# Autodesk Inventor assembly: Drivetrain Assembled
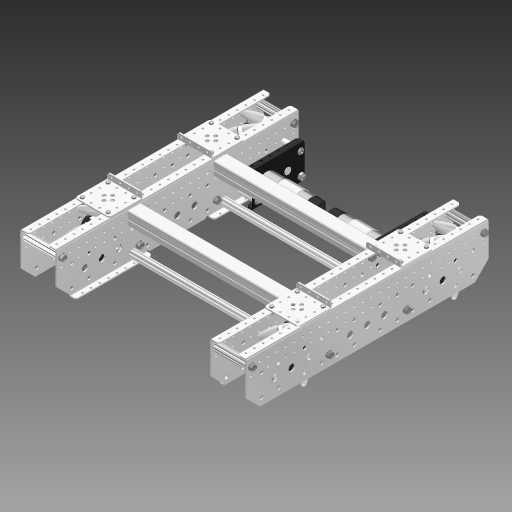
[picture p0: Inventor's stored thumbnail of the model, 512x512]
Saved by Autodesk Inventor 2024 (Build 280153000, 153)
## iProperties
Created: 2023-11-08
Part Number: Drivetrain Assembled
Document SubType Name: Assembly
Designer: Calvin
Author: Calvin
## Documents named in this file (25)
- C:\Users\Calvin\Desktop\CAD\Alt\ironChefsCAD\Drivetrain\Drivetrain Assembled.iam
- C:\Users\Calvin\Desktop\CAD\Alt\ironChefsCAD\Drivetrain\Parts\TileRunner 17 Inside Plate.ipt
- C:\Users\Calvin\Desktop\CAD\Alt\ironChefsCAD\Drivetrain\Parts\TileRunner 17 Outside Plate.ipt
- C:\Users\Calvin\Desktop\CAD\Alt\ironChefsCAD\Drivetrain\Parts\63mm Churro.ipt
- C:\Users\Calvin\Desktop\CAD\Alt\ironChefsCAD\Drivetrain\Parts\FHTS 0.25-20-0.75_FHTS 0.25-20-G-0.75-C.ipt
- C:\Users\Calvin\Desktop\CAD\Alt\ironChefsCAD\Drivetrain\Parts\TileRunner 17 4x4 Hole Bracket.ipt
- C:\Users\Calvin\Desktop\CAD\Alt\ironChefsCAD\Drivetrain\Parts\6-32 Nylock Nut_90631A007.ipt
- C:\Users\Calvin\Desktop\CAD\Alt\ironChefsCAD\Drivetrain\Parts\6-32 x 0500 HHCS_93075A148.ipt
- C:\Users\Calvin\Desktop\CAD\Alt\ironChefsCAD\Drivetrain\Parts\11.250in Peanut.ipt
- C:\Users\Calvin\Desktop\CAD\Alt\ironChefsCAD\Drivetrain\Parts\11.250in Churro.ipt
- C:\Users\Calvin\Desktop\CAD\Alt\ironChefsCAD\Drivetrain\Parts\PicoBox Uno Plate.ipt
- C:\Users\Calvin\Desktop\CAD\Alt\ironChefsCAD\Drivetrain\Parts\PicoBox Spacer.ipt
- C:\Users\Calvin\Desktop\CAD\Alt\ironChefsCAD\Drivetrain\Parts\14-20 x 1.625 BHCS_92949A837.ipt
- C:\Users\Calvin\Desktop\CAD\Alt\ironChefsCAD\Drivetrain\Parts\14-20 NyLock thin - Mcm 90566A029_90566A029.ipt
- C:\Users\Calvin\Desktop\CAD\Alt\ironChefsCAD\Drivetrain\Parts\6mm x 12mm Flanged -Mcm 7804K142_7804K142.ipt
- C:\Users\Calvin\Desktop\CAD\Alt\ironChefsCAD\Drivetrain\Parts\6mm D-Shaft 100mm.ipt
- C:\Users\Calvin\Desktop\CAD\Alt\ironChefsCAD\Drivetrain\Parts\am-2964 NeveRest.ipt
- C:\Users\Calvin\Desktop\CAD\Alt\ironChefsCAD\Drivetrain\Parts\40T 32DP 20PA With 6mm Bore Nub Gear.ipt
- C:\Users\Calvin\Desktop\CAD\Alt\ironChefsCAD\Drivetrain\Parts\am-3215 6mmD Double Boss Nub.ipt
- C:\Users\Calvin\Desktop\CAD\Alt\ironChefsCAD\Drivetrain\Parts\10-32 x 0.25 Set Screw Cup Point.ipt
- C:\Users\Calvin\Desktop\CAD\Alt\ironChefsCAD\Drivetrain\Parts\M3x0.5x6mm SHCS_91290A111.ipt
- C:\Users\Calvin\Desktop\CAD\Alt\ironChefsCAD\Drivetrain\Parts\406 right wheel.iam
- C:\Users\Calvin\Desktop\CAD\Alt\ironChefsCAD\Drivetrain\Parts\6-32 x 1250 HHCS_93075A544.ipt
- C:\Users\Calvin\Desktop\CAD\Alt\ironChefsCAD\Drivetrain\Parts\9mmt x 6.15mm ID Aluminum Spacer AluminumSpacers.com MAS13-6-9.ipt
- C:\Users\Calvin\Desktop\CAD\Alt\ironChefsCAD\Drivetrain\Parts\.594t x .257 ID Aluminum Spacer AluminumSpacers.com AS38-14-38.ipt
## Components (158 placed, 24 different names)
1. TileRunner 17 Inside Plate:1 — Insert:4, Angle:1, Flush:2, Symmetry:1, Insert:67, Angle:3, Insert:73, Insert:119, Angle:5
2. TileRunner 17 Outside Plate:1 — Insert:3, Angle:1, Insert:11, Insert:12, Insert:13, Flush:1, Insert:145, Insert:148
3. 63mm Churro:1 — Insert:1, Insert:2, Insert:3, Insert:4
4. FHTS 0.25-20-0.75_FHTS 0.25-20-G-0.75-C:1 — Insert:1
5. FHTS 0.25-20-0.75_FHTS 0.25-20-G-0.75-C:2 — Insert:2
6. 63mm Churro:2 — Insert:11
7. FHTS 0.25-20-0.75_FHTS 0.25-20-G-0.75-C:3
8. FHTS 0.25-20-0.75_FHTS 0.25-20-G-0.75-C:4
9. 63mm Churro:3 — Insert:12
10. FHTS 0.25-20-0.75_FHTS 0.25-20-G-0.75-C:5
11. FHTS 0.25-20-0.75_FHTS 0.25-20-G-0.75-C:6
12. 63mm Churro:4 — Insert:13
13. FHTS 0.25-20-0.75_FHTS 0.25-20-G-0.75-C:7
14. FHTS 0.25-20-0.75_FHTS 0.25-20-G-0.75-C:8
15. TileRunner 17 Inside Plate:2 — Flush:2, Symmetry:1, Insert:68, Angle:4, Mate:5, Insert:74, Insert:120, Angle:6
16. TileRunner 17 Outside Plate:2 — Flush:1, Flush:12, Mate:2, Mate:3, Mate:4, Insert:146, Insert:147
17. 63mm Churro:5
18. FHTS 0.25-20-0.75_FHTS 0.25-20-G-0.75-C:9
19. FHTS 0.25-20-0.75_FHTS 0.25-20-G-0.75-C:10
20. 63mm Churro:6
21. FHTS 0.25-20-0.75_FHTS 0.25-20-G-0.75-C:11
22. FHTS 0.25-20-0.75_FHTS 0.25-20-G-0.75-C:12
23. 63mm Churro:7
24. FHTS 0.25-20-0.75_FHTS 0.25-20-G-0.75-C:13
25. FHTS 0.25-20-0.75_FHTS 0.25-20-G-0.75-C:14
26. 63mm Churro:8
27. FHTS 0.25-20-0.75_FHTS 0.25-20-G-0.75-C:15
28. FHTS 0.25-20-0.75_FHTS 0.25-20-G-0.75-C:16
29. TileRunner 17 4x4 Hole Bracket:1 — Insert:31, Insert:32, Insert:33, Insert:34, Flush:3, Flush:5, Flush:9, Symmetry:3
30. 6-32 Nylock Nut_90631A007:1 — Insert:27
31. 6-32 x 0500 HHCS_93075A148:1 — Insert:27, Insert:31
32. 6-32 Nylock Nut_90631A007:2
33. 6-32 x 0500 HHCS_93075A148:2 — Insert:32
34. 6-32 Nylock Nut_90631A007:3
35. 6-32 x 0500 HHCS_93075A148:3 — Insert:33
36. 6-32 Nylock Nut_90631A007:4
37. 6-32 x 0500 HHCS_93075A148:4 — Insert:34
38. TileRunner 17 4x4 Hole Bracket:2 — Flush:3, Flush:5, Flush:7, Flush:8, Symmetry:2, Mate:3, Mate:4, Symmetry:3
39. 6-32 Nylock Nut_90631A007:5
40. 6-32 x 0500 HHCS_93075A148:5
41. 6-32 Nylock Nut_90631A007:6
42. 6-32 x 0500 HHCS_93075A148:6
43. 6-32 Nylock Nut_90631A007:7
44. 6-32 x 0500 HHCS_93075A148:7
45. 6-32 Nylock Nut_90631A007:8
46. 6-32 x 0500 HHCS_93075A148:8
47. TileRunner 17 4x4 Hole Bracket:3 — Flush:4, Flush:6, Flush:9
48. 6-32 Nylock Nut_90631A007:9
49. 6-32 x 0500 HHCS_93075A148:9
50. 6-32 Nylock Nut_90631A007:10
51. 6-32 x 0500 HHCS_93075A148:10
52. 6-32 Nylock Nut_90631A007:11
53. 6-32 x 0500 HHCS_93075A148:11
54. 6-32 Nylock Nut_90631A007:12
55. 6-32 x 0500 HHCS_93075A148:12
56. TileRunner 17 4x4 Hole Bracket:4 — Flush:4, Flush:6, Flush:7, Flush:8, Symmetry:2
57. 6-32 Nylock Nut_90631A007:13
58. 6-32 x 0500 HHCS_93075A148:13
59. 6-32 Nylock Nut_90631A007:14
60. 6-32 x 0500 HHCS_93075A148:14
61. 6-32 Nylock Nut_90631A007:15
62. 6-32 x 0500 HHCS_93075A148:15
63. 6-32 Nylock Nut_90631A007:16
64. 6-32 x 0500 HHCS_93075A148:16
65. FHTS 0.25-20-0.75_FHTS 0.25-20-G-0.75-C:17 — Insert:59
66. FHTS 0.25-20-0.75_FHTS 0.25-20-G-0.75-C:18 — Insert:60
67. 11.250in Peanut:1 — Insert:59, Insert:60, Insert:61, Insert:62, Insert:67, Angle:3, Mate:5
68. FHTS 0.25-20-0.75_FHTS 0.25-20-G-0.75-C:19 — Insert:62
69. FHTS 0.25-20-0.75_FHTS 0.25-20-G-0.75-C:20 — Insert:61
70. FHTS 0.25-20-0.75_FHTS 0.25-20-G-0.75-C:21
71. FHTS 0.25-20-0.75_FHTS 0.25-20-G-0.75-C:22
72. 11.250in Peanut:2 — Insert:68, Angle:4
73. FHTS 0.25-20-0.75_FHTS 0.25-20-G-0.75-C:23
74. FHTS 0.25-20-0.75_FHTS 0.25-20-G-0.75-C:24
75. 11.250in Churro:1 — Insert:69, Insert:70, Insert:73
76. FHTS 0.25-20-0.75_FHTS 0.25-20-G-0.75-C:25 — Insert:70
77. FHTS 0.25-20-0.75_FHTS 0.25-20-G-0.75-C:26 — Insert:69
78. 11.250in Churro:2 — Insert:74
79. FHTS 0.25-20-0.75_FHTS 0.25-20-G-0.75-C:27
80. FHTS 0.25-20-0.75_FHTS 0.25-20-G-0.75-C:28
81. PicoBox Uno Plate:1 — Insert:76, Insert:84, Insert:85, Insert:86, Insert:87, Mate:6, Insert:88, Insert:90, Angle:5
82. PicoBox Spacer:2 — Insert:75, Insert:76
83. 14-20 x 1.625 BHCS_92949A837:4 — Insert:75, Insert:77
84. 6mm x 12mm Flanged -Mcm 7804K142_7804K142:1 — Insert:89, Insert:90, Mate:11
85. 6mm x 12mm Flanged -Mcm 7804K142_7804K142:2 — Insert:96
86. 6mm D-Shaft 100mm:1 — Insert:89, Mate:9
87. am-2964 NeveRest:1 — Insert:87, Mate:6, Mate:10
88. 10-32 x 0.25 Set Screw Cup Point:2 — Insert:92
89. am-3215 6mmD Double Boss Nub:2 — Insert:92, Insert:93, Mate:7, Insert:96
90. 40T 32DP 20PA With 6mm Bore Nub Gear:2 — Insert:91, Insert:93, Mate:7, Flush:13, Mate:9, Mate:11
91. 14-20 NyLock thin - Mcm 90566A029_90566A029:1 — Insert:77
92. PicoBox Spacer:3 — Insert:119
93. 14-20 x 1.625 BHCS_92949A837:5 — Insert:84
94. 14-20 NyLock thin - Mcm 90566A029_90566A029:2
95. PicoBox Spacer:4
96. 14-20 x 1.625 BHCS_92949A837:6 — Insert:85
97. 14-20 NyLock thin - Mcm 90566A029_90566A029:3
98. PicoBox Spacer:5
99. 14-20 x 1.625 BHCS_92949A837:7 — Insert:86
100. 14-20 NyLock thin - Mcm 90566A029_90566A029:4
101. M3x0.5x6mm SHCS_91290A111:1 — Insert:88
102. am-3215 6mmD Double Boss Nub:3
103. 40T 32DP 20PA With 6mm Bore Nub Gear:3 — Flush:13, Mate:10
104. 6-32 x 0500 HHCS_93075A148:21 — Insert:91
105. 6-32 x 0500 HHCS_93075A148:22
106. PicoBox Uno Plate:2 — Angle:6
107. PicoBox Spacer:6 — Insert:120
108. 14-20 x 1.625 BHCS_92949A837:8
109. 6mm x 12mm Flanged -Mcm 7804K142_7804K142:3
110. 6mm x 12mm Flanged -Mcm 7804K142_7804K142:4
111. 6mm D-Shaft 100mm:2
112. am-2964 NeveRest:2
113. 10-32 x 0.25 Set Screw Cup Point:3
114. am-3215 6mmD Double Boss Nub:4
115. 40T 32DP 20PA With 6mm Bore Nub Gear:4
116. 6-32 x 0500 HHCS_93075A148:23
117. M3x0.5x6mm SHCS_91290A111:2
118. 14-20 NyLock thin - Mcm 90566A029_90566A029:5
119. PicoBox Spacer:7
120. 14-20 x 1.625 BHCS_92949A837:9
121. 14-20 NyLock thin - Mcm 90566A029_90566A029:6
122. PicoBox Spacer:8
123. 14-20 x 1.625 BHCS_92949A837:10
124. 14-20 NyLock thin - Mcm 90566A029_90566A029:7
125. PicoBox Spacer:9
126. 14-20 x 1.625 BHCS_92949A837:11
127. 14-20 NyLock thin - Mcm 90566A029_90566A029:8
128. am-3215 6mmD Double Boss Nub:5
129. 40T 32DP 20PA With 6mm Bore Nub Gear:5
130. 6-32 x 0500 HHCS_93075A148:24
131. 406 right wheel:1 [sub-assembly] — Insert:121, Insert:122, Mate:18, Insert:126
132. 6mm x 12mm Flanged -Mcm 7804K142_7804K142:5 — Insert:125, Insert:145
133. am-3215 6mmD Double Boss Nub:6 — Insert:122, Mate:18, Insert:123, Insert:124
134. 10-32 x 0.25 Set Screw Cup Point:4 — Insert:123
135. 9mmt x 6.15mm ID Aluminum Spacer AluminumSpacers.com MAS13-6-9:1 — Insert:124
136. 6-32 x 1250 HHCS_93075A544:3 — Insert:121
137. .594t x .257 ID Aluminum Spacer AluminumSpacers.com AS38-14-38:1 — Insert:125, Insert:126
138. 406 right wheel:2 [sub-assembly]
139. 6mm x 12mm Flanged -Mcm 7804K142_7804K142:6 — Insert:146
140. am-3215 6mmD Double Boss Nub:7
141. 10-32 x 0.25 Set Screw Cup Point:5
142. 9mmt x 6.15mm ID Aluminum Spacer AluminumSpacers.com MAS13-6-9:2
143. 6-32 x 1250 HHCS_93075A544:4
144. .594t x .257 ID Aluminum Spacer AluminumSpacers.com AS38-14-38:2
145. 406 right wheel:3 [sub-assembly]
146. 6mm x 12mm Flanged -Mcm 7804K142_7804K142:7 — Insert:148
147. am-3215 6mmD Double Boss Nub:8
148. 10-32 x 0.25 Set Screw Cup Point:6
149. 9mmt x 6.15mm ID Aluminum Spacer AluminumSpacers.com MAS13-6-9:3
150. 6-32 x 1250 HHCS_93075A544:5
151. .594t x .257 ID Aluminum Spacer AluminumSpacers.com AS38-14-38:3
152. 406 right wheel:4 [sub-assembly]
153. 6mm x 12mm Flanged -Mcm 7804K142_7804K142:8 — Insert:147
154. am-3215 6mmD Double Boss Nub:9
155. 10-32 x 0.25 Set Screw Cup Point:7
156. 9mmt x 6.15mm ID Aluminum Spacer AluminumSpacers.com MAS13-6-9:4
157. 6-32 x 1250 HHCS_93075A544:6
158. .594t x .257 ID Aluminum Spacer AluminumSpacers.com AS38-14-38:4
## Relationships (189: Insert 148, Mate 20, Flush 12, Angle 6, Symmetry 3)
- Insert:1 (2.286 mm): 63mm Churro:1 ↔ FHTS 0.25-20-0.75_FHTS 0.25-20-G-0.75-C:1
- Insert:2 (2.286 mm): 63mm Churro:1 ↔ FHTS 0.25-20-0.75_FHTS 0.25-20-G-0.75-C:2
- Insert:3: TileRunner 17 Outside Plate:1 ↔ 63mm Churro:1
- Insert:4: TileRunner 17 Inside Plate:1 ↔ 63mm Churro:1
- Angle:1 (0 deg): TileRunner 17 Inside Plate:1 ↔ TileRunner 17 Outside Plate:1
- [Insert] (2.286 mm): 63mm Churro:2 ↔ FHTS 0.25-20-0.75_FHTS 0.25-20-G-0.75-C:3
- [Insert] (2.286 mm): 63mm Churro:2 ↔ FHTS 0.25-20-0.75_FHTS 0.25-20-G-0.75-C:4
- [Insert] (2.286 mm): 63mm Churro:3 ↔ FHTS 0.25-20-0.75_FHTS 0.25-20-G-0.75-C:5
- [Insert] (2.286 mm): 63mm Churro:3 ↔ FHTS 0.25-20-0.75_FHTS 0.25-20-G-0.75-C:6
- [Insert] (2.286 mm): 63mm Churro:4 ↔ FHTS 0.25-20-0.75_FHTS 0.25-20-G-0.75-C:7
- [Insert] (2.286 mm): 63mm Churro:4 ↔ FHTS 0.25-20-0.75_FHTS 0.25-20-G-0.75-C:8
- Insert:11: TileRunner 17 Outside Plate:1 ↔ 63mm Churro:2
- Insert:12: TileRunner 17 Outside Plate:1 ↔ 63mm Churro:3
- Insert:13: TileRunner 17 Outside Plate:1 ↔ 63mm Churro:4
- [Insert] (2.286 mm): 63mm Churro:5 ↔ FHTS 0.25-20-0.75_FHTS 0.25-20-G-0.75-C:9
- [Insert] (2.286 mm): 63mm Churro:5 ↔ FHTS 0.25-20-0.75_FHTS 0.25-20-G-0.75-C:10
- [Insert]: TileRunner 17 Outside Plate:2 ↔ 63mm Churro:5
- [Insert]: TileRunner 17 Inside Plate:2 ↔ 63mm Churro:5
- [Angle] (0 deg): TileRunner 17 Inside Plate:2 ↔ TileRunner 17 Outside Plate:2
- [Insert] (2.286 mm): 63mm Churro:6 ↔ FHTS 0.25-20-0.75_FHTS 0.25-20-G-0.75-C:11
- [Insert] (2.286 mm): 63mm Churro:6 ↔ FHTS 0.25-20-0.75_FHTS 0.25-20-G-0.75-C:12
- [Insert] (2.286 mm): 63mm Churro:7 ↔ FHTS 0.25-20-0.75_FHTS 0.25-20-G-0.75-C:13
- [Insert] (2.286 mm): 63mm Churro:7 ↔ FHTS 0.25-20-0.75_FHTS 0.25-20-G-0.75-C:14
- [Insert] (2.286 mm): 63mm Churro:8 ↔ FHTS 0.25-20-0.75_FHTS 0.25-20-G-0.75-C:15
- [Insert] (2.286 mm): 63mm Churro:8 ↔ FHTS 0.25-20-0.75_FHTS 0.25-20-G-0.75-C:16
- [Insert]: TileRunner 17 Outside Plate:2 ↔ 63mm Churro:6
- [Insert]: TileRunner 17 Outside Plate:2 ↔ 63mm Churro:7
- [Insert]: TileRunner 17 Outside Plate:2 ↔ 63mm Churro:8
- Flush:1: TileRunner 17 Outside Plate:1 ↔ TileRunner 17 Outside Plate:2
- Flush:2: TileRunner 17 Inside Plate:1 ↔ TileRunner 17 Inside Plate:2
- Symmetry:1: TileRunner 17 Inside Plate:1 ↔ TileRunner 17 Inside Plate:2
- Flush:12: TileRunner 17 Outside Plate:2
- Mate:2 (50.8 mm): TileRunner 17 Outside Plate:2
- Insert:27 (-4.572 mm): 6-32 Nylock Nut_90631A007:1 ↔ 6-32 x 0500 HHCS_93075A148:1
- [Insert] (-4.572 mm): 6-32 Nylock Nut_90631A007:2 ↔ 6-32 x 0500 HHCS_93075A148:2
- [Insert] (-4.572 mm): 6-32 Nylock Nut_90631A007:3 ↔ 6-32 x 0500 HHCS_93075A148:3
- [Insert] (-4.572 mm): 6-32 Nylock Nut_90631A007:4 ↔ 6-32 x 0500 HHCS_93075A148:4
- Insert:31: TileRunner 17 4x4 Hole Bracket:1 ↔ 6-32 x 0500 HHCS_93075A148:1
- Insert:32: TileRunner 17 4x4 Hole Bracket:1 ↔ 6-32 x 0500 HHCS_93075A148:2
- Insert:33: TileRunner 17 4x4 Hole Bracket:1 ↔ 6-32 x 0500 HHCS_93075A148:3
- Insert:34: TileRunner 17 4x4 Hole Bracket:1 ↔ 6-32 x 0500 HHCS_93075A148:4
- [Insert] (-4.572 mm): 6-32 Nylock Nut_90631A007:5 ↔ 6-32 x 0500 HHCS_93075A148:5
- [Insert] (-4.572 mm): 6-32 Nylock Nut_90631A007:6 ↔ 6-32 x 0500 HHCS_93075A148:6
- [Insert] (-4.572 mm): 6-32 Nylock Nut_90631A007:7 ↔ 6-32 x 0500 HHCS_93075A148:7
- [Insert] (-4.572 mm): 6-32 Nylock Nut_90631A007:8 ↔ 6-32 x 0500 HHCS_93075A148:8
- [Insert]: TileRunner 17 4x4 Hole Bracket:2 ↔ 6-32 x 0500 HHCS_93075A148:5
- [Insert]: TileRunner 17 4x4 Hole Bracket:2 ↔ 6-32 x 0500 HHCS_93075A148:6
- [Insert]: TileRunner 17 4x4 Hole Bracket:2 ↔ 6-32 x 0500 HHCS_93075A148:7
- [Insert]: TileRunner 17 4x4 Hole Bracket:2 ↔ 6-32 x 0500 HHCS_93075A148:8
- [Insert] (-4.572 mm): 6-32 Nylock Nut_90631A007:9 ↔ 6-32 x 0500 HHCS_93075A148:9
- [Insert] (-4.572 mm): 6-32 Nylock Nut_90631A007:10 ↔ 6-32 x 0500 HHCS_93075A148:10
- [Insert] (-4.572 mm): 6-32 Nylock Nut_90631A007:11 ↔ 6-32 x 0500 HHCS_93075A148:11
- [Insert] (-4.572 mm): 6-32 Nylock Nut_90631A007:12 ↔ 6-32 x 0500 HHCS_93075A148:12
- [Insert]: TileRunner 17 4x4 Hole Bracket:3 ↔ 6-32 x 0500 HHCS_93075A148:9
- [Insert]: TileRunner 17 4x4 Hole Bracket:3 ↔ 6-32 x 0500 HHCS_93075A148:10
- [Insert]: TileRunner 17 4x4 Hole Bracket:3 ↔ 6-32 x 0500 HHCS_93075A148:11
- [Insert]: TileRunner 17 4x4 Hole Bracket:3 ↔ 6-32 x 0500 HHCS_93075A148:12
- [Insert] (-4.572 mm): 6-32 Nylock Nut_90631A007:13 ↔ 6-32 x 0500 HHCS_93075A148:13
- [Insert] (-4.572 mm): 6-32 Nylock Nut_90631A007:14 ↔ 6-32 x 0500 HHCS_93075A148:14
- [Insert] (-4.572 mm): 6-32 Nylock Nut_90631A007:15 ↔ 6-32 x 0500 HHCS_93075A148:15
- [Insert] (-4.572 mm): 6-32 Nylock Nut_90631A007:16 ↔ 6-32 x 0500 HHCS_93075A148:16
- [Insert]: TileRunner 17 4x4 Hole Bracket:4 ↔ 6-32 x 0500 HHCS_93075A148:13
- [Insert]: TileRunner 17 4x4 Hole Bracket:4 ↔ 6-32 x 0500 HHCS_93075A148:14
- [Insert]: TileRunner 17 4x4 Hole Bracket:4 ↔ 6-32 x 0500 HHCS_93075A148:15
- [Insert]: TileRunner 17 4x4 Hole Bracket:4 ↔ 6-32 x 0500 HHCS_93075A148:16
- Flush:3: TileRunner 17 4x4 Hole Bracket:1 ↔ TileRunner 17 4x4 Hole Bracket:2
- Flush:4: TileRunner 17 4x4 Hole Bracket:3 ↔ TileRunner 17 4x4 Hole Bracket:4
- Flush:5: TileRunner 17 4x4 Hole Bracket:1 ↔ TileRunner 17 4x4 Hole Bracket:2
- Flush:6: TileRunner 17 4x4 Hole Bracket:3 ↔ TileRunner 17 4x4 Hole Bracket:4
- Flush:7: TileRunner 17 4x4 Hole Bracket:2 ↔ TileRunner 17 4x4 Hole Bracket:4
- Flush:8: TileRunner 17 4x4 Hole Bracket:2 ↔ TileRunner 17 4x4 Hole Bracket:4
- Flush:9: TileRunner 17 4x4 Hole Bracket:1 ↔ TileRunner 17 4x4 Hole Bracket:3
- Symmetry:2: TileRunner 17 4x4 Hole Bracket:2 ↔ TileRunner 17 4x4 Hole Bracket:4
- Mate:3: TileRunner 17 Outside Plate:2 ↔ TileRunner 17 4x4 Hole Bracket:2
- Mate:4: TileRunner 17 Outside Plate:2 ↔ TileRunner 17 4x4 Hole Bracket:2
- Symmetry:3: TileRunner 17 4x4 Hole Bracket:1 ↔ TileRunner 17 4x4 Hole Bracket:2
- Insert:59 (2.286 mm): FHTS 0.25-20-0.75_FHTS 0.25-20-G-0.75-C:17 ↔ 11.250in Peanut:1
- Insert:60 (2.286 mm): FHTS 0.25-20-0.75_FHTS 0.25-20-G-0.75-C:18 ↔ 11.250in Peanut:1
- Insert:61 (2.286 mm): 11.250in Peanut:1 ↔ FHTS 0.25-20-0.75_FHTS 0.25-20-G-0.75-C:20
- Insert:62 (2.286 mm): 11.250in Peanut:1 ↔ FHTS 0.25-20-0.75_FHTS 0.25-20-G-0.75-C:19
- [Insert] (2.286 mm): FHTS 0.25-20-0.75_FHTS 0.25-20-G-0.75-C:21 ↔ 11.250in Peanut:2
- [Insert] (2.286 mm): FHTS 0.25-20-0.75_FHTS 0.25-20-G-0.75-C:22 ↔ 11.250in Peanut:2
- [Insert] (2.286 mm): 11.250in Peanut:2 ↔ FHTS 0.25-20-0.75_FHTS 0.25-20-G-0.75-C:24
- [Insert] (2.286 mm): 11.250in Peanut:2 ↔ FHTS 0.25-20-0.75_FHTS 0.25-20-G-0.75-C:23
- Insert:67: TileRunner 17 Inside Plate:1 ↔ 11.250in Peanut:1
- Angle:3 (0 deg): TileRunner 17 Inside Plate:1 ↔ 11.250in Peanut:1
- Insert:68: TileRunner 17 Inside Plate:2 ↔ 11.250in Peanut:2
- Angle:4 (0 deg): TileRunner 17 Inside Plate:2 ↔ 11.250in Peanut:2
- Mate:5: TileRunner 17 Inside Plate:2 ↔ 11.250in Peanut:1
- Insert:69 (2.286 mm): 11.250in Churro:1 ↔ FHTS 0.25-20-0.75_FHTS 0.25-20-G-0.75-C:26
- Insert:70 (2.286 mm): 11.250in Churro:1 ↔ FHTS 0.25-20-0.75_FHTS 0.25-20-G-0.75-C:25
- [Insert] (2.286 mm): 11.250in Churro:2 ↔ FHTS 0.25-20-0.75_FHTS 0.25-20-G-0.75-C:28
- [Insert] (2.286 mm): 11.250in Churro:2 ↔ FHTS 0.25-20-0.75_FHTS 0.25-20-G-0.75-C:27
- Insert:73: TileRunner 17 Inside Plate:1 ↔ 11.250in Churro:1
- Insert:74: TileRunner 17 Inside Plate:2 ↔ 11.250in Churro:2
- Insert:75 (2.286 mm): PicoBox Spacer:2 ↔ 14-20 x 1.625 BHCS_92949A837:4
- Insert:76: PicoBox Uno Plate:1 ↔ PicoBox Spacer:2
- Insert:77 (1.778 mm): 14-20 x 1.625 BHCS_92949A837:4 ↔ 14-20 NyLock thin - Mcm 90566A029_90566A029:1
- [Insert] (2.286 mm): PicoBox Spacer:3 ↔ 14-20 x 1.625 BHCS_92949A837:5
- [Insert] (1.778 mm): 14-20 x 1.625 BHCS_92949A837:5 ↔ 14-20 NyLock thin - Mcm 90566A029_90566A029:2
- [Insert] (2.286 mm): PicoBox Spacer:4 ↔ 14-20 x 1.625 BHCS_92949A837:6
- [Insert] (1.778 mm): 14-20 x 1.625 BHCS_92949A837:6 ↔ 14-20 NyLock thin - Mcm 90566A029_90566A029:3
- [Insert] (2.286 mm): PicoBox Spacer:5 ↔ 14-20 x 1.625 BHCS_92949A837:7
- [Insert] (1.778 mm): 14-20 x 1.625 BHCS_92949A837:7 ↔ 14-20 NyLock thin - Mcm 90566A029_90566A029:4
- Insert:84: PicoBox Uno Plate:1 ↔ 14-20 x 1.625 BHCS_92949A837:5
- Insert:85: PicoBox Uno Plate:1 ↔ 14-20 x 1.625 BHCS_92949A837:6
- Insert:86: PicoBox Uno Plate:1 ↔ 14-20 x 1.625 BHCS_92949A837:7
- Insert:87: PicoBox Uno Plate:1 ↔ am-2964 NeveRest:1
- Mate:6: PicoBox Uno Plate:1 ↔ am-2964 NeveRest:1
- Insert:88: PicoBox Uno Plate:1 ↔ M3x0.5x6mm SHCS_91290A111:1
- Insert:89: 6mm x 12mm Flanged -Mcm 7804K142_7804K142:1 ↔ 6mm D-Shaft 100mm:1
- Insert:90: PicoBox Uno Plate:1 ↔ 6mm x 12mm Flanged -Mcm 7804K142_7804K142:1
- Insert:91: 40T 32DP 20PA With 6mm Bore Nub Gear:2 ↔ 6-32 x 0500 HHCS_93075A148:21
- Insert:92: 10-32 x 0.25 Set Screw Cup Point:2 ↔ am-3215 6mmD Double Boss Nub:2
- Insert:93: am-3215 6mmD Double Boss Nub:2 ↔ 40T 32DP 20PA With 6mm Bore Nub Gear:2
- Mate:7: am-3215 6mmD Double Boss Nub:2 ↔ 40T 32DP 20PA With 6mm Bore Nub Gear:2
- [Insert]: 40T 32DP 20PA With 6mm Bore Nub Gear:3 ↔ 6-32 x 0500 HHCS_93075A148:22
- [Insert]: am-3215 6mmD Double Boss Nub:3 ↔ 40T 32DP 20PA With 6mm Bore Nub Gear:3
- [Mate]: am-3215 6mmD Double Boss Nub:3 ↔ 40T 32DP 20PA With 6mm Bore Nub Gear:3
- Flush:13: 40T 32DP 20PA With 6mm Bore Nub Gear:2 ↔ 40T 32DP 20PA With 6mm Bore Nub Gear:3
- Mate:9: 6mm D-Shaft 100mm:1 ↔ 40T 32DP 20PA With 6mm Bore Nub Gear:2
- Mate:10: am-2964 NeveRest:1 ↔ 40T 32DP 20PA With 6mm Bore Nub Gear:3
- Mate:11 (9 mm): 6mm x 12mm Flanged -Mcm 7804K142_7804K142:1 ↔ 40T 32DP 20PA With 6mm Bore Nub Gear:2
- Insert:96: 6mm x 12mm Flanged -Mcm 7804K142_7804K142:2 ↔ am-3215 6mmD Double Boss Nub:2
- [Insert] (2.286 mm): PicoBox Spacer:6 ↔ 14-20 x 1.625 BHCS_92949A837:8
- [Insert]: PicoBox Uno Plate:2 ↔ PicoBox Spacer:6
- [Insert] (1.778 mm): 14-20 x 1.625 BHCS_92949A837:8 ↔ 14-20 NyLock thin - Mcm 90566A029_90566A029:5
- [Insert] (2.286 mm): PicoBox Spacer:7 ↔ 14-20 x 1.625 BHCS_92949A837:9
- [Insert] (1.778 mm): 14-20 x 1.625 BHCS_92949A837:9 ↔ 14-20 NyLock thin - Mcm 90566A029_90566A029:6
- [Insert] (2.286 mm): PicoBox Spacer:8 ↔ 14-20 x 1.625 BHCS_92949A837:10
- [Insert] (1.778 mm): 14-20 x 1.625 BHCS_92949A837:10 ↔ 14-20 NyLock thin - Mcm 90566A029_90566A029:7
- [Insert] (2.286 mm): PicoBox Spacer:9 ↔ 14-20 x 1.625 BHCS_92949A837:11
- [Insert] (1.778 mm): 14-20 x 1.625 BHCS_92949A837:11 ↔ 14-20 NyLock thin - Mcm 90566A029_90566A029:8
- [Insert]: PicoBox Uno Plate:2 ↔ 14-20 x 1.625 BHCS_92949A837:9
- [Insert]: PicoBox Uno Plate:2 ↔ 14-20 x 1.625 BHCS_92949A837:10
- [Insert]: PicoBox Uno Plate:2 ↔ 14-20 x 1.625 BHCS_92949A837:11
- [Insert]: PicoBox Uno Plate:2 ↔ am-2964 NeveRest:2
- [Mate]: PicoBox Uno Plate:2 ↔ am-2964 NeveRest:2
- [Insert]: PicoBox Uno Plate:2 ↔ M3x0.5x6mm SHCS_91290A111:2
- [Insert]: 6mm x 12mm Flanged -Mcm 7804K142_7804K142:3 ↔ 6mm D-Shaft 100mm:2
- [Insert]: PicoBox Uno Plate:2 ↔ 6mm x 12mm Flanged -Mcm 7804K142_7804K142:3
- [Insert]: 40T 32DP 20PA With 6mm Bore Nub Gear:4 ↔ 6-32 x 0500 HHCS_93075A148:23
- [Insert]: 10-32 x 0.25 Set Screw Cup Point:3 ↔ am-3215 6mmD Double Boss Nub:4
- [Insert]: am-3215 6mmD Double Boss Nub:4 ↔ 40T 32DP 20PA With 6mm Bore Nub Gear:4
- [Mate]: am-3215 6mmD Double Boss Nub:4 ↔ 40T 32DP 20PA With 6mm Bore Nub Gear:4
- [Insert]: 40T 32DP 20PA With 6mm Bore Nub Gear:5 ↔ 6-32 x 0500 HHCS_93075A148:24
- [Insert]: am-3215 6mmD Double Boss Nub:5 ↔ 40T 32DP 20PA With 6mm Bore Nub Gear:5
- [Mate]: am-3215 6mmD Double Boss Nub:5 ↔ 40T 32DP 20PA With 6mm Bore Nub Gear:5
- [Flush]: 40T 32DP 20PA With 6mm Bore Nub Gear:4 ↔ 40T 32DP 20PA With 6mm Bore Nub Gear:5
- [Mate]: 6mm D-Shaft 100mm:2 ↔ 40T 32DP 20PA With 6mm Bore Nub Gear:4
- [Mate]: am-2964 NeveRest:2 ↔ 40T 32DP 20PA With 6mm Bore Nub Gear:5
- [Mate] (9 mm): 6mm x 12mm Flanged -Mcm 7804K142_7804K142:3 ↔ 40T 32DP 20PA With 6mm Bore Nub Gear:4
- [Insert]: 6mm x 12mm Flanged -Mcm 7804K142_7804K142:4 ↔ am-3215 6mmD Double Boss Nub:4
- Insert:119: TileRunner 17 Inside Plate:1 ↔ PicoBox Spacer:3
- Angle:5 (0 deg): TileRunner 17 Inside Plate:1 ↔ PicoBox Uno Plate:1
- Insert:120: TileRunner 17 Inside Plate:2 ↔ PicoBox Spacer:6
- Angle:6 (0 deg): TileRunner 17 Inside Plate:2 ↔ PicoBox Uno Plate:2
- Insert:121: 406 right wheel:1 ↔ 6-32 x 1250 HHCS_93075A544:3
- Insert:122: 406 right wheel:1 ↔ am-3215 6mmD Double Boss Nub:6
- Mate:18: 406 right wheel:1 ↔ am-3215 6mmD Double Boss Nub:6
- Insert:123: am-3215 6mmD Double Boss Nub:6 ↔ 10-32 x 0.25 Set Screw Cup Point:4
- Insert:124: am-3215 6mmD Double Boss Nub:6 ↔ 9mmt x 6.15mm ID Aluminum Spacer AluminumSpacers.com MAS13-6-9:1
- Insert:125: 6mm x 12mm Flanged -Mcm 7804K142_7804K142:5 ↔ .594t x .257 ID Aluminum Spacer AluminumSpacers.com AS38-14-38:1
- Insert:126: 406 right wheel:1 ↔ .594t x .257 ID Aluminum Spacer AluminumSpacers.com AS38-14-38:1
- [Insert]: 406 right wheel:2 ↔ 6-32 x 1250 HHCS_93075A544:4
- [Insert]: 406 right wheel:2 ↔ am-3215 6mmD Double Boss Nub:7
- [Mate]: 406 right wheel:2 ↔ am-3215 6mmD Double Boss Nub:7
- [Insert]: am-3215 6mmD Double Boss Nub:7 ↔ 10-32 x 0.25 Set Screw Cup Point:5
- [Insert]: am-3215 6mmD Double Boss Nub:7 ↔ 9mmt x 6.15mm ID Aluminum Spacer AluminumSpacers.com MAS13-6-9:2
- [Insert]: 6mm x 12mm Flanged -Mcm 7804K142_7804K142:6 ↔ .594t x .257 ID Aluminum Spacer AluminumSpacers.com AS38-14-38:2
- [Insert]: 406 right wheel:2 ↔ .594t x .257 ID Aluminum Spacer AluminumSpacers.com AS38-14-38:2
- [Insert]: 406 right wheel:3 ↔ 6-32 x 1250 HHCS_93075A544:5
- [Insert]: 406 right wheel:3 ↔ am-3215 6mmD Double Boss Nub:8
- [Mate]: 406 right wheel:3 ↔ am-3215 6mmD Double Boss Nub:8
- [Insert]: am-3215 6mmD Double Boss Nub:8 ↔ 10-32 x 0.25 Set Screw Cup Point:6
- [Insert]: am-3215 6mmD Double Boss Nub:8 ↔ 9mmt x 6.15mm ID Aluminum Spacer AluminumSpacers.com MAS13-6-9:3
- [Insert]: 6mm x 12mm Flanged -Mcm 7804K142_7804K142:7 ↔ .594t x .257 ID Aluminum Spacer AluminumSpacers.com AS38-14-38:3
- [Insert]: 406 right wheel:3 ↔ .594t x .257 ID Aluminum Spacer AluminumSpacers.com AS38-14-38:3
- [Insert]: 406 right wheel:4 ↔ 6-32 x 1250 HHCS_93075A544:6
- [Insert]: 406 right wheel:4 ↔ am-3215 6mmD Double Boss Nub:9
- [Mate]: 406 right wheel:4 ↔ am-3215 6mmD Double Boss Nub:9
- [Insert]: am-3215 6mmD Double Boss Nub:9 ↔ 10-32 x 0.25 Set Screw Cup Point:7
- [Insert]: am-3215 6mmD Double Boss Nub:9 ↔ 9mmt x 6.15mm ID Aluminum Spacer AluminumSpacers.com MAS13-6-9:4
- [Insert]: 6mm x 12mm Flanged -Mcm 7804K142_7804K142:8 ↔ .594t x .257 ID Aluminum Spacer AluminumSpacers.com AS38-14-38:4
- [Insert]: 406 right wheel:4 ↔ .594t x .257 ID Aluminum Spacer AluminumSpacers.com AS38-14-38:4
- Insert:145: TileRunner 17 Outside Plate:1 ↔ 6mm x 12mm Flanged -Mcm 7804K142_7804K142:5
- Insert:146: TileRunner 17 Outside Plate:2 ↔ 6mm x 12mm Flanged -Mcm 7804K142_7804K142:6
- Insert:147: TileRunner 17 Outside Plate:2 ↔ 6mm x 12mm Flanged -Mcm 7804K142_7804K142:8
- Insert:148: TileRunner 17 Outside Plate:1 ↔ 6mm x 12mm Flanged -Mcm 7804K142_7804K142:7
## Named parameters: d5_d0 = 2.286 mm, d6_d1 = 2.286 mm, d7_d0 = 2.286 mm, d8_d1 = 2.286 mm, d9_d0 = 2.286 mm, d10_d1 = 2.286 mm, d14_d0 = 2.286 mm, d15_d1 = 2.286 mm, d16_d2 = 0 mm, d17_d3 = 0 mm, d18_d4 = 0 deg, d19_d5_d0 = 2.286 mm, d20_d6_d1 = 2.286 mm, d21_d7_d0 = 2.286 mm, d22_d8_d1 = 2.286 mm, d23_d9_d0 = 2.286 mm, d24_d10_d1 = 2.286 mm, d25_d11 = 0 mm, d26_d12 = 0 mm, d27_d13 = 0 mm, d33_d32 = -4.572 mm, d34_d32 = -4.572 mm, d35_d32 = -4.572 mm, d40_d32 = -4.572 mm, d41_d33_d32 = -4.572 mm, d42_d34_d32 = -4.572 mm, d43_d35_d32 = -4.572 mm, d44_d36 = 0 mm, d45_d37 = 0 mm, d46_d38 = 0 mm, d47_d39 = 0 mm, d48_d32 = -4.572 mm, d49_d33_d32 = -4.572 mm, d50_d34_d32 = -4.572 mm, d51_d35_d32 = -4.572 mm, d52_d36 = 0 mm, d53_d37 = 0 mm, d54_d38 = 0 mm, d55_d39 = 0 mm, d56_d32 = -4.572 mm, d57_d33_d32 = -4.572 mm, d58_d34_d32 = -4.572 mm, d59_d35_d32 = -4.572 mm, d60_d36 = 0 mm, d61_d37 = 0 mm, d62_d38 = 0 mm, d63_d39 = 0 mm, d79_d75 = 2.286 mm, d80_d76 = 2.286 mm, d81_d77 = 2.286 mm, d82_d78 = 2.286 mm, d90_d88 = 2.286 mm, d91_d89 = 2.286 mm, d100_d96 = 2.286 mm, d101_d99 = 1.778 mm, d102_d96 = 2.286 mm, d103_d99 = 1.778 mm, d104_d96 = 2.286 mm, d105_d99 = 1.778 mm, d120_d116 = 0 mm, d121_d118 = 0 mm, d122_d119 = 0 mm, d132_d96 = 2.286 mm, d133_d97 = 0 mm, d134_d99 = 1.778 mm, d135_d100_d96 = 2.286 mm, d136_d101_d99 = 1.778 mm, d137_d102_d96 = 2.286 mm, d138_d103_d99 = 1.778 mm, d139_d104_d96 = 2.286 mm, d140_d105_d99 = 1.778 mm, d141_d106 = 0 mm, d142_d107 = 0 mm, d143_d108 = 0 mm, d144_d109 = 0 mm, d145_d110 = 0 mm, d146_d111 = 0 mm, d147_d114 = 0 mm, d148_d115 = 0 mm, d149_d116 = 0 mm, d150_d117 = 0 mm, d151_d118 = 0 mm, d152_d119 = 0 mm, d153_d120_d116 = 0 mm, d154_d121_d118 = 0 mm, d155_d122_d119 = 0 mm, d156_d127 = 0 mm, d157_d128 = 0 mm, d158_d129 = 0 mm, d159_d130 = 9 mm, d160_d131 = 0 mm, d172_d165 = 0 mm, d173_d166 = 0 mm, d174_d167 = 0 mm, d175_d168 = 0 mm, d176_d169 = 0 mm, d177_d170 = 0 mm, d178_d171 = 0 mm, d179_d165 = 0 mm, d180_d166 = 0 mm, d181_d167 = 0 mm, d182_d168 = 0 mm, d183_d169 = 0 mm, d184_d170 = 0 mm, d185_d171 = 0 mm, d186_d165 = 0 mm, d187_d166 = 0 mm, d188_d167 = 0 mm, d189_d168 = 0 mm, d190_d169 = 0 mm, d191_d170 = 0 mm, d192_d171 = 0 mm
